# Autodesk Inventor assembly: PDRHN30
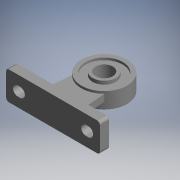
[picture p0: Inventor's stored thumbnail of the model, 180x180]
Saved by Autodesk Inventor 2017.3 (Build 213256000, 256)
## iProperties
Category: PARTsolutions
Company: MISUMI
Part Number: PDRHN30
Catalog Web Link: www.cadenas.de
Description: PDRH,PDRHN-Ball Bearing Units -High-Centered Pillow Type-
Vendor: MISUMI
Document SubType Name: Assembly
Designer: partserver
Manufacturer: MISUMI
Mass: 268.984 g
Surface Area: 527.366 cm^2
Volume: 268.984 cm^3
Density: 1 g/cm^3
Title: PDRHN30
Author: Cadenas PARTsolutions
Comments: Ball Bearing Units -High-Centered Pillow Type-
PSOL_IDENT_0: {$CADENAS_DATA\23d-libs\misumi\metric\12_bearing_holders\pdrh_asmtab.prj},174 {VTYP=3D},{STYP=ASSTAB
PSOL_IDENT_1: },{NB=PDRHN30},{LINA=PDRHN30},{NN=PDRH,PDRHN},{DATE=11.12.2019 10:07:02},{GEOMDATE=02.12.2019 09:15:
PSOL_IDENT_2: 31},{VERSION=},{LINEID=60},{WBVAR=TS},{WBNUMERIC=}  {NB=PDRHN30},{LINA=PDRHN30},{KT=DUMMY},{PN=PDRHN
PSOL_IDENT_3: 30},{TYPE=PDRHN},{MATH=Cast Iron Class No.30},{MATB=52100 Bearing Steel},{MATRS=Nitrile Rubber},{MAT
PSOL_IDENT_4: SS=4137 Alloy Steel},{PRECISION=JIS B 1558/JIS B 1514/JIS B 1559},{OT=-15 ~+100},{TS=2},{TSALG='1','
PSOL_IDENT_5: Lubrication Type' , '2','Oil-Free Type'},{D=30},{JIS=UC206D1},{H=90},{L=165},{L1=120},{A=50},{DD1=21
PSOL_IDENT_6: },{DD=17},{TT=16},{H1=130},{B=38.1},{S=15.9},{CR=19.5},{COR=11.30},{M1=M6x0.75},{MD=6},{MPITCH=0.75}
PSOL_IDENT_7: ,{ML=8},{MASS=1800},{RLD1=80},{RLD2=65},{RLD3=40.8},{LD1=28},{LD2=4.0},{LD3=2},{G1=28.5},{G2=12.0},{
PSOL_IDENT_8: G3=50},{R1=11},{R2=5},{NCL=1.9},{KCL=17.2},{PPATH=pdrh/pdrh_asmtpl.prj}
NB: PDRHN30
NN: PDRH,PDRHN
NT: Ball Bearing Units -High-Centered Pillow Type-
NBSYN: $PN.
LINA: PDRHN30
CATALOG: Misumi
PN: PDRHN30
TYPE: PDRHN
MATH: Cast Iron Class No.30
MATB: 52100 Bearing Steel
MATRS: Nitrile Rubber
MATSS: 4137 Alloy Steel
PRECISION: JIS B 1558/JIS B 1514/JIS B 1559
OT: -15 ~+100
TS: Oil-Free Type
D: 30
JIS: UC206D1
H: 90
L: 165
L1: 120
A: 50
DD1: 21
DD: 17
TT: 16
H1: 130
B: 38.1
S: 15.9
CR: 19.5
COR: 11.3
M1: M6x0.75
MASS: 1800
PPATH: pdrh/pdrh_asmtpl.prj
SUPPLIER: MISUMI
ARTICLENO: PDRHN30
BOMINFO: PDRHN30
CREATOR: CADENAS GmbH
## Documents named in this file (3)
- e:\temp\worker_19\temp\exporttempdir_4596_40_0wU4X\format_0\PDRHN30.iam
- e:\temp\worker_19\temp\exporttempdir_4596_40_0wU4X\format_0\PDRHN30_b.ipt
- e:\temp\worker_19\temp\exporttempdir_4596_40_0wU4X\format_0\SET-SCREW6-8.ipt
## Components (3 placed, 2 different names)
1. PDRHN30_b:1 — CP1_XY@1 <-> CP_XY@2, CP1_Z@1 <-> CP_Z@2, CP1_YZ@1 <-> CP_YZ@2, CP2_XY@1 <-> CP_XY@3, CP2_Z@1 <-> CP_Z@3, CP2_YZ@1 <-> CP_YZ@3
2. SET-SCREW6-8:1 — CP1_XY@1 <-> CP_XY@2, CP1_Z@1 <-> CP_Z@2, CP1_YZ@1 <-> CP_YZ@2
3. SET-SCREW6-8:2 — CP2_XY@1 <-> CP_XY@3, CP2_Z@1 <-> CP_Z@3, CP2_YZ@1 <-> CP_YZ@3
## Relationships (6: Mate 4, Angle 2)
- CP1_XY@1 <-> CP_XY@2 [Mate]: PDRHN30_b:1 ↔ SET-SCREW6-8:1
- CP1_Z@1 <-> CP_Z@2 [Mate]: PDRHN30_b:1 ↔ SET-SCREW6-8:1
- CP1_YZ@1 <-> CP_YZ@2 [Angle] (0 deg): PDRHN30_b:1 ↔ SET-SCREW6-8:1
- CP2_XY@1 <-> CP_XY@3 [Mate]: PDRHN30_b:1 ↔ SET-SCREW6-8:2
- CP2_Z@1 <-> CP_Z@3 [Mate]: PDRHN30_b:1 ↔ SET-SCREW6-8:2
- CP2_YZ@1 <-> CP_YZ@3 [Angle] (0 deg): PDRHN30_b:1 ↔ SET-SCREW6-8:2
